# Autodesk Inventor assembly: UNLHEP-14-01-A-003_ChuckW4modules
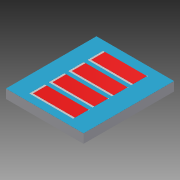
[picture p0: Inventor's stored thumbnail of the model, 180x180]
Saved by Autodesk Inventor 2013 (Build 170138000, 138)
## iProperties
Created: 2014-01-06
Part Number: UNLHEP-14-01-A-003_ChuckW4modules
Document SubType Name: Assembly
Designer: Frank Meier
Project: UNL Pixel Phase I
Author: Frank Meier
Revision Number: 00
## Documents named in this file (4)
- C:\Users\Frank Meier\Documents\Inventor\Delvotec-Saugplatte\UNLHEP-14-01-A-003_ChuckW4modules.iam
- C:\Users\Frank Meier\Documents\Inventor\Delvotec-Saugplatte\UNLHEP-14-01-P-001_ModuleChuck.ipt
- C:\Users\Frank Meier\Documents\Inventor\Delvotec-Saugplatte\UNLHEP-14-01-P-006_SensorMock.ipt
- C:\Users\Frank Meier\Documents\Inventor\Delvotec-Saugplatte\UNLHEP-14-01-P-005_ModuleStencil.ipt
## Components (3 placed, 3 different names)
1. UNLHEP-14-P-01-001_ModuleChuck:1 — Fluchtend:1, Fluchtend:2, Fluchtend:3, Fluchtend:4, Fluchtend:5
2. UNLHEP-14-P-01-006_SensorMock:1 — Fluchtend:1, Fluchtend:2, Fluchtend:3
3. UNLHEP-14-P-01-005_ModuleStencil:1 — Fluchtend:4, Fluchtend:5
## Relationships (5: Flush 5)
- Fluchtend:1 [Flush]: UNLHEP-14-P-01-001_ModuleChuck:1 ↔ UNLHEP-14-P-01-006_SensorMock:1
- Fluchtend:2 [Flush] (27.6 mm): UNLHEP-14-P-01-001_ModuleChuck:1 ↔ UNLHEP-14-P-01-006_SensorMock:1
- Fluchtend:3 [Flush] (14.42 mm): UNLHEP-14-P-01-001_ModuleChuck:1 ↔ UNLHEP-14-P-01-006_SensorMock:1
- Fluchtend:4 [Flush]: UNLHEP-14-P-01-001_ModuleChuck:1 ↔ UNLHEP-14-P-01-005_ModuleStencil:1
- Fluchtend:5 [Flush]: UNLHEP-14-P-01-001_ModuleChuck:1 ↔ UNLHEP-14-P-01-005_ModuleStencil:1
